# Autodesk Inventor assembly: assembled
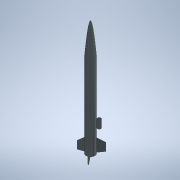
[picture p0: Inventor's stored thumbnail of the model, 180x180]
Saved by Autodesk Inventor 2020 (Build 240168000, 168)
## iProperties
Created: 2021-01-23
Part Number: assembled
Document SubType Name: Assembly
Designer: 0x6f736f646f
Author: 0x6f736f646f
## Documents named in this file (5)
- C:\Users\0x6f736f646f\OneDrive\Documents\Inventor\Nakuja project\assembled.iam
- C:\Users\0x6f736f646f\OneDrive\Documents\Inventor\Nakuja project\nose.ipt
- C:\Users\0x6f736f646f\OneDrive\Documents\Inventor\Nakuja project\payloadchamber.ipt
- C:\Users\0x6f736f646f\OneDrive\Documents\Inventor\Nakuja project\tail.ipt
- C:\Users\0x6f736f646f\OneDrive\Documents\Inventor\Nakuja project\launchlug.ipt
## Components (4 placed, 4 different names)
1. nose:1 — Insert:1
2. payloadchamber:1 — Mate:1, Insert:1, Mate:2
3. tail:1 — Mate:1, Mate:2, Mate:3, Mate:4, Mate:5
4. launchlug:1 — Mate:3, Mate:4, Mate:5
## Relationships (6: Mate 5, Insert 1)
- Mate:1: payloadchamber:1 ↔ tail:1
- Insert:1: nose:1 ↔ payloadchamber:1
- Mate:2: payloadchamber:1 ↔ tail:1
- Mate:3 (23.6 mm): tail:1 ↔ launchlug:1
- Mate:4: tail:1 ↔ launchlug:1
- Mate:5 (90 mm): tail:1 ↔ launchlug:1
